# Autodesk Inventor assembly: element_R
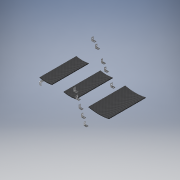
[picture p0: Inventor's stored thumbnail of the model, 180x180]
Saved by Autodesk Inventor 2018.1 (Build 221171000, 171)
## iProperties
Created: 2017-10-22
Part Number: element_R
Material: 一般
Document SubType Name: Assembly
Designer: ku_sk
Author: ku_sk
## Documents named in this file (4)
- D:\ku_sk\ドキュメント\Inventor\KS-15_Aero_CAD\type4\F-wing\parts\element_R.iam
- D:\ku_sk\ドキュメント\Inventor\KS-15_Aero_CAD\type4\F-wing\parts\element_1.ipt
- D:\ku_sk\ドキュメント\Inventor\KS-15_Aero_CAD\type4\F-wing\parts\element_2.ipt
- D:\ku_sk\ドキュメント\Inventor\KS-15_Aero_CAD\type4\F-wing\parts\element_clip.ipt
## Components (15 placed, 3 different names)
1. element_1:1
2. element_2:1 — フラッシュ:1
3. element_2:2
4. element_clip:1 — フラッシュ:1
5. element_clip:2
6. element_clip:3
7. element_clip:4
8. element_clip:5
9. element_clip:6
10. element_clip:7
11. element_clip:8
12. element_clip:9
13. element_clip:10
14. element_clip:11
15. element_clip:12
## Relationships (1: Flush 1)
- フラッシュ:1 [Flush]: element_2:1 ↔ element_clip:1
